# Autodesk Inventor assembly: 2020-04-02-10-50001-LED_Splitter
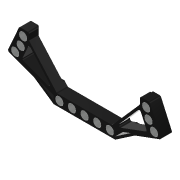
[picture p0: Inventor's stored thumbnail of the model, 180x180]
Saved by Autodesk Inventor 2020 (Build 240168000, 168)
## iProperties
Created: 2020-11-04
Part Number: 2020-04-02-10-50001-LED_Splitter
Document SubType Name: Assembly
Designer: eunde
Author: eunde
## Documents named in this file (3)
- Y:\Technik\Technik 2020\04 - Electronics\02 - Digital Circuits\10 - MSWC\2020-04-02-10-50001-LED_Splitter.iam
- Y:\Technik\Technik 2020\04 - Electronics\02 - Digital Circuits\10 - MSWC\2020-04-02-10-10501-LED_Splitter.ipt
- Y:\Technik\Technik 2020\04 - Electronics\02 - Digital Circuits\10 - MSWC\2020-04-02-10-10701-LED_Acryl_Glas.ipt
## Components (12 placed, 2 different names)
1. 2020-04-02-10-10501-LED_Splitter:1 — Mate:1, Mate:2, Mate:3, Mate:4, Mate:5, Mate:6, Mate:7, Mate:8, Mate:9, Mate:10, Mate:11, Flush:1, Flush:2, Flush:3, Flush:4, Flush:5, Flush:6, Flush:7, Flush:8, Flush:9, Flush:10, Flush:11
2. 2020-04-02-10-10701-LED_Acryl_Glas:1 — Mate:2, Flush:2
3. 2020-04-02-10-10701-LED_Acryl_Glas:2 — Mate:8, Flush:8
4. 2020-04-02-10-10701-LED_Acryl_Glas:3 — Mate:3, Flush:3
5. 2020-04-02-10-10701-LED_Acryl_Glas:4 — Mate:5, Flush:5
6. 2020-04-02-10-10701-LED_Acryl_Glas:5 — Mate:4, Flush:4
7. 2020-04-02-10-10701-LED_Acryl_Glas:6 — Mate:6, Flush:6
8. 2020-04-02-10-10701-LED_Acryl_Glas:7 — Mate:7, Flush:7
9. 2020-04-02-10-10701-LED_Acryl_Glas:8 — Mate:9, Flush:9
10. 2020-04-02-10-10701-LED_Acryl_Glas:9 — Mate:11, Flush:11
11. 2020-04-02-10-10701-LED_Acryl_Glas:10 — Mate:10, Flush:10
12. 2020-04-02-10-10701-LED_Acryl_Glas:11 — Mate:1, Flush:1
## Relationships (22: Mate 11, Flush 11)
- Mate:1: 2020-04-02-10-10501-LED_Splitter:1 ↔ 2020-04-02-10-10701-LED_Acryl_Glas:11
- Mate:2: 2020-04-02-10-10501-LED_Splitter:1 ↔ 2020-04-02-10-10701-LED_Acryl_Glas:1
- Mate:3: 2020-04-02-10-10501-LED_Splitter:1 ↔ 2020-04-02-10-10701-LED_Acryl_Glas:3
- Mate:4: 2020-04-02-10-10501-LED_Splitter:1 ↔ 2020-04-02-10-10701-LED_Acryl_Glas:5
- Mate:5: 2020-04-02-10-10501-LED_Splitter:1 ↔ 2020-04-02-10-10701-LED_Acryl_Glas:4
- Mate:6: 2020-04-02-10-10501-LED_Splitter:1 ↔ 2020-04-02-10-10701-LED_Acryl_Glas:6
- Mate:7: 2020-04-02-10-10501-LED_Splitter:1 ↔ 2020-04-02-10-10701-LED_Acryl_Glas:7
- Mate:8: 2020-04-02-10-10501-LED_Splitter:1 ↔ 2020-04-02-10-10701-LED_Acryl_Glas:2
- Mate:9: 2020-04-02-10-10501-LED_Splitter:1 ↔ 2020-04-02-10-10701-LED_Acryl_Glas:8
- Mate:10: 2020-04-02-10-10501-LED_Splitter:1 ↔ 2020-04-02-10-10701-LED_Acryl_Glas:10
- Mate:11: 2020-04-02-10-10501-LED_Splitter:1 ↔ 2020-04-02-10-10701-LED_Acryl_Glas:9
- Flush:1: 2020-04-02-10-10501-LED_Splitter:1 ↔ 2020-04-02-10-10701-LED_Acryl_Glas:11
- Flush:2: 2020-04-02-10-10501-LED_Splitter:1 ↔ 2020-04-02-10-10701-LED_Acryl_Glas:1
- Flush:3: 2020-04-02-10-10501-LED_Splitter:1 ↔ 2020-04-02-10-10701-LED_Acryl_Glas:3
- Flush:4: 2020-04-02-10-10501-LED_Splitter:1 ↔ 2020-04-02-10-10701-LED_Acryl_Glas:5
- Flush:5: 2020-04-02-10-10501-LED_Splitter:1 ↔ 2020-04-02-10-10701-LED_Acryl_Glas:4
- Flush:6: 2020-04-02-10-10501-LED_Splitter:1 ↔ 2020-04-02-10-10701-LED_Acryl_Glas:6
- Flush:7: 2020-04-02-10-10501-LED_Splitter:1 ↔ 2020-04-02-10-10701-LED_Acryl_Glas:7
- Flush:8: 2020-04-02-10-10501-LED_Splitter:1 ↔ 2020-04-02-10-10701-LED_Acryl_Glas:2
- Flush:9: 2020-04-02-10-10501-LED_Splitter:1 ↔ 2020-04-02-10-10701-LED_Acryl_Glas:8
- Flush:10: 2020-04-02-10-10501-LED_Splitter:1 ↔ 2020-04-02-10-10701-LED_Acryl_Glas:10
- Flush:11: 2020-04-02-10-10501-LED_Splitter:1 ↔ 2020-04-02-10-10701-LED_Acryl_Glas:9
